# Autodesk Inventor assembly: DJB_Case_Rev-4
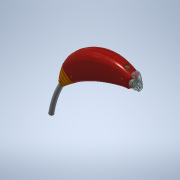
[picture p0: Inventor's stored thumbnail of the model, 180x180]
Saved by Autodesk Inventor 2020 (Build 240168000, 168)
## iProperties
Created: 2020-01-07
Part Number: DJB_Case_Rev-4
Document SubType Name: Assembly
Designer: Mark.Neilson
Mass: 9.37315 g
Surface Area: 88.3333 cm^2
Volume: 9.29368 cm^3
Density: 1.00855 g/cm^3
Author: Mark.Neilson
## Documents named in this file (14)
- C:\Users\alex.lynch\Nextcloud\Documents\UCSD OpenSpeech\CAD\DJB parametric CAD files\200226\DJB_Case_Rev-4.iam
- C:\Users\alex.lynch\Nextcloud\Documents\UCSD OpenSpeech\CAD\DJB parametric CAD files\200226\Socket_CS44_10.iam
- C:\Users\alex.lynch\Nextcloud\Documents\UCSD OpenSpeech\CAD\DJB parametric CAD files\200226\DJB_Case_Rev-4-Bot.ipt
- C:\Users\alex.lynch\Nextcloud\Documents\UCSD OpenSpeech\CAD\DJB parametric CAD files\200226\DJB_Case_Rev-4-Top.ipt
- C:\Users\alex.lynch\Nextcloud\Documents\UCSD OpenSpeech\CAD\DJB parametric CAD files\200226\99A-1097044000.ipt
- C:\Users\alex.lynch\Nextcloud\Documents\UCSD OpenSpeech\CAD\DJB parametric CAD files\200226\DJB_Case_Rev-4-Chassis_R_1.ipt
- C:\Users\alex.lynch\Nextcloud\Documents\UCSD OpenSpeech\CAD\DJB parametric CAD files\200226\DJB_Case_Rev-4-Chassis_L_1.ipt
- C:\Users\alex.lynch\Nextcloud\Documents\UCSD OpenSpeech\CAD\DJB parametric CAD files\200226\djb_v2_rigid.ipt
- C:\Users\alex.lynch\Nextcloud\Documents\UCSD OpenSpeech\CAD\DJB parametric CAD files\200226\DJB_v2_Flex.iam
- C:\Users\alex.lynch\Nextcloud\Documents\UCSD OpenSpeech\CAD\DJB parametric CAD files\200226\1-47a0001_023x263R.ipt
- C:\Users\alex.lynch\Nextcloud\Documents\UCSD OpenSpeech\CAD\DJB parametric CAD files\200226\1-47a0311_023x245R.ipt
- C:\Users\alex.lynch\Nextcloud\Documents\UCSD OpenSpeech\CAD\DJB parametric CAD files\200226\DJB_Case_Rev-4-StrainRelief_1.ipt
- C:\Users\alex.lynch\Nextcloud\Documents\UCSD OpenSpeech\CAD\DJB parametric CAD files\200226\PowerCord.ipt
- C:\Users\alex.lynch\Nextcloud\Documents\UCSD OpenSpeech\CAD\DJB parametric CAD files\200226\1-RIE_CS44 Connetor-0.040Shielded.iam
## Components (16 placed, 13 different names)
1. DJB_Case_Rev-4-Bot:1 — Mate:15, Mate:16, Mate:17, Mate:18, Insert:3, Mate:28, Insert:4
2. DJB_Case_Rev-4-Top:1 — Mate:20, Mate:22, Flush:1
3. DJB_Case_Rev-4-Chassis_R_1:1 — Mate:6, Mate:7, Mate:8, Mate:9, Mate:10, Mate:11, Angle:1, Insert:1
4. djb_v2_rigid.ipt:5 — Insert:2, Angle:1
5. Socket_CS44_10:1 [sub-assembly] — Insert:1, Insert:2
6. DJB_v2_Flex.iam:6 [sub-assembly]
7. 99A-1097044000:1 — Mate:6, Mate:7, Mate:8
8. 99A-1097044000:2 — Mate:9, Mate:10, Mate:11
9. DJB_Case_Rev-4-Chassis_L_1:1
10. DJB_Case_Rev-4-StrainRelief_1:1 — Mate:25, Mate:26, Mate:27, Flush:1, Insert:4
11. 1-47a0311_023x245R:1 — Mate:15, Mate:16
12. 1-47a0311_023x245R:2 — Mate:17, Mate:18
13. 1-47a0001_023x263R:1 — Mate:20
14. 1-47a0001_023x263R:2 — Mate:22
15. PowerCord:1 — Mate:25, Mate:26, Mate:27
16. 1-RIE_CS44 Connetor-0.040Shielded:1 [sub-assembly] — Insert:3, Mate:28
## Relationships (27: Mate 21, Insert 4, Angle 1, Flush 1)
- Insert:1 (0.0254 mm): DJB_Case_Rev-4-Chassis_R_1:1 ↔ Socket_CS44_10:1
- Mate:6: DJB_Case_Rev-4-Chassis_R_1:1 ↔ 99A-1097044000:1
- Mate:7: DJB_Case_Rev-4-Chassis_R_1:1 ↔ 99A-1097044000:1
- Mate:8: DJB_Case_Rev-4-Chassis_R_1:1 ↔ 99A-1097044000:1
- Mate:9: DJB_Case_Rev-4-Chassis_R_1:1 ↔ 99A-1097044000:2
- Mate:10: DJB_Case_Rev-4-Chassis_R_1:1 ↔ 99A-1097044000:2
- Mate:11: DJB_Case_Rev-4-Chassis_R_1:1 ↔ 99A-1097044000:2
- [Mate]: djb_v2_rigid.ipt:5 ↔ DJB_v2_Flex.iam:6
- [Mate] (0.0127 mm): djb_v2_rigid.ipt:5 ↔ DJB_v2_Flex.iam:6
- [Mate] (0.0127 mm): djb_v2_rigid.ipt:5 ↔ DJB_v2_Flex.iam:6
- Mate:15: DJB_Case_Rev-4-Bot:1 ↔ 1-47a0311_023x245R:1
- Mate:16: DJB_Case_Rev-4-Bot:1 ↔ 1-47a0311_023x245R:1
- Mate:17: DJB_Case_Rev-4-Bot:1 ↔ 1-47a0311_023x245R:2
- Mate:18: DJB_Case_Rev-4-Bot:1 ↔ 1-47a0311_023x245R:2
- [Mate]: DJB_Case_Rev-4-Top:1 ↔ 1-47a0001_023x263R:1
- Mate:20: DJB_Case_Rev-4-Top:1 ↔ 1-47a0001_023x263R:1
- [Mate]: DJB_Case_Rev-4-Top:1 ↔ 1-47a0001_023x263R:2
- Mate:22: DJB_Case_Rev-4-Top:1 ↔ 1-47a0001_023x263R:2
- Insert:2: djb_v2_rigid.ipt:5 ↔ Socket_CS44_10:1
- Angle:1 (0 deg): DJB_Case_Rev-4-Chassis_R_1:1 ↔ djb_v2_rigid.ipt:5
- Mate:25: DJB_Case_Rev-4-StrainRelief_1:1 ↔ PowerCord:1
- Mate:26: DJB_Case_Rev-4-StrainRelief_1:1 ↔ PowerCord:1
- Mate:27: DJB_Case_Rev-4-StrainRelief_1:1 ↔ PowerCord:1
- Insert:3: DJB_Case_Rev-4-Bot:1 ↔ 1-RIE_CS44 Connetor-0.040Shielded:1
- Mate:28: DJB_Case_Rev-4-Bot:1 ↔ 1-RIE_CS44 Connetor-0.040Shielded:1
- Flush:1: DJB_Case_Rev-4-Top:1 ↔ DJB_Case_Rev-4-StrainRelief_1:1
- Insert:4: DJB_Case_Rev-4-Bot:1 ↔ DJB_Case_Rev-4-StrainRelief_1:1
